# Autodesk Inventor assembly: Assembly_GaragenBox
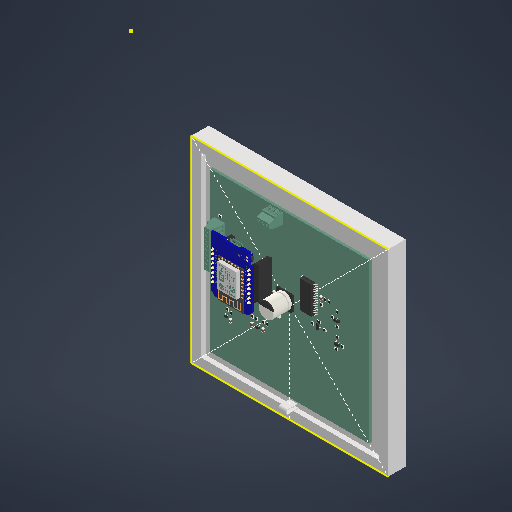
[picture p0: Inventor's stored thumbnail of the model, 512x512]
Saved by Autodesk Inventor 2027 (Build 310192000, 192)
## iProperties
Created: 2026-02-04
Part Number: Assembly_GaragenBox
Document SubType Name: Assembly
Designer: schoe
Author: schoe
## Documents named in this file (3)
- E:\GitHub\garage-project\pcb\Garage-Box-Project\Assembly_GaragenBox.iam
- E:\GitHub\garage-project\pcb\Garage-Box-Project\Box_with_PCBRefernce.ipt
- E:\GitHub\garage-project\pcb\Garage-Box-Project\Clipper.ipt
## Components (2 placed, 2 different names)
1. Box_with_PCBRefernce:1 — Mate:1, Mate:2, Flush:6
2. Clipper:1 — Mate:1, Mate:2, Flush:6
## Relationships (3: Mate 2, Flush 1)
- Mate:1: Box_with_PCBRefernce:1 ↔ Clipper:1
- Mate:2: Box_with_PCBRefernce:1 ↔ Clipper:1
- Flush:6: Box_with_PCBRefernce:1 ↔ Clipper:1
